# Autodesk Inventor assembly: Motor Med Chain gear
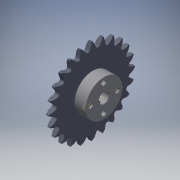
[picture p0: Inventor's stored thumbnail of the model, 180x180]
Saved by Autodesk Inventor 2016 (Build 200138000, 138)
## iProperties
Created: 2015-12-15
Part Number: Motor Med Chain gear
Document SubType Name: Assembly
Designer: TimB
Author: TimB
## Documents named in this file (4)
- C:\Users\TimB\Documents\GitHub\phi_robotics\3d-models\FTC_Tetrix_KOP_Block_Party\Tim Bloot Designs\JAr JaR Bot\Motor Med Chain gear.iam
- C:\Users\TimB\Documents\GitHub\phi_robotics\3d-models\FTC_Tetrix_KOP_Block_Party\Tetrix_Kit_FTC\Autodesk Inventor Files\tetrix_maxle_lock.iam
- C:\Users\TimB\Documents\GitHub\phi_robotics\3d-models\FTC_Tetrix_KOP_Block_Party\Tetrix_Kit_FTC\Autodesk Inventor Files\tetrix_screw.ipt
- C:\Users\TimB\Documents\GitHub\phi_robotics\3d-models\FTC_Tetrix_KOP_Block_Party\Tetrix_Kit_FTC\Autodesk Inventor Files\tetrix_chain_gear-24t.ipt
## Components (4 placed, 3 different names)
1. tetrix_maxle_lock:1 [sub-assembly] — Rigid:1
2. tetrix_screw:1 — Rigid:3
3. tetrix_screw:2 — Rigid:2
4. tetrix_chain_gear-24t:1 — Rigid:1, Rigid:2, Rigid:3
## Relationships (3: WeldJoint 3)
- Rigid:1 [WeldJoint]: tetrix_maxle_lock:1 ↔ tetrix_chain_gear-24t:1
- Rigid:2 [WeldJoint]: tetrix_screw:2 ↔ tetrix_chain_gear-24t:1
- Rigid:3 [WeldJoint]: tetrix_screw:1 ↔ tetrix_chain_gear-24t:1
